# Autodesk Inventor assembly: Leg3DOF-Front-Left
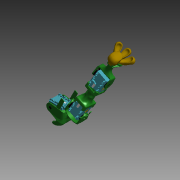
[picture p0: Inventor's stored thumbnail of the model, 180x180]
Saved by Autodesk Inventor 2016 (Build 200138000, 138)
## iProperties
Created: 2015-03-02
Part Number: Leg3DOF-Front-Left
Document SubType Name: Assembly
Designer: Henke
Author: Henke
## Documents named in this file (5)
- G:\Study_and_Projekts\KEX_robotik\CAD\Leg3DOF-Front-Left.iam
- G:\Study_and_Projekts\KEX_robotik\CAD\Servo with wheel.iam
- G:\Study_and_Projekts\KEX_robotik\CAD\StraightConnector.ipt
- G:\Study_and_Projekts\KEX_robotik\CAD\HipConnector-Front.ipt
- G:\Study_and_Projekts\KEX_robotik\CAD\Foot assembly.iam
## Components (6 placed, 4 different names)
1. Servo with wheel:1 [sub-assembly] — Rotational:2
2. Servo with wheel:2 [sub-assembly] — Mate:7, Mate:8, Mate:9, Rotational:1
3. Servo with wheel:3 [sub-assembly] — Mate:10, Mate:11, Flush:1, Mate:12, Mate:15
4. StraightConnector:1 — Mate:7, Mate:8, Mate:9, Mate:10, Mate:11, Flush:1
5. Foot assembly:1 [sub-assembly] — Mate:12, Mate:15
6. HipConnector-Front:1 — Rotational:1, Rotational:2
## Relationships (10: Mate 7, RevoluteJoint 2, Flush 1)
- Mate:7: Servo with wheel:2 ↔ StraightConnector:1
- Mate:8: Servo with wheel:2 ↔ StraightConnector:1
- Mate:9: Servo with wheel:2 ↔ StraightConnector:1
- Mate:10: Servo with wheel:3 ↔ StraightConnector:1
- Mate:11: Servo with wheel:3 ↔ StraightConnector:1
- Flush:1: Servo with wheel:3 ↔ StraightConnector:1
- Mate:12: Servo with wheel:3 ↔ Foot assembly:1
- Mate:15: Servo with wheel:3 ↔ Foot assembly:1
- Rotational:1 [RevoluteJoint]: Servo with wheel:2 ↔ HipConnector-Front:1
- Rotational:2 [RevoluteJoint]: Servo with wheel:1 ↔ HipConnector-Front:1
